# Autodesk Inventor assembly: Caster
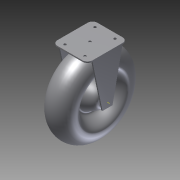
[picture p0: Inventor's stored thumbnail of the model, 180x180]
Saved by Autodesk Inventor 2012 (Build 160160000, 160)
## iProperties
Created: 2011-10-20
Part Number: Caster
Document SubType Name: Assembly
Designer: robotics
Author: robotics
## Documents named in this file (3)
- C:\Users\robotics\Dropbox\CAD Inventor\Preseason Projects\Cart Competition Cart\Team 2374\Caster.iam
- C:\Users\robotics\Dropbox\CAD Inventor\Preseason Projects\Cart Competition Cart\Team 2374\Caster2.ipt
- C:\Users\robotics\Dropbox\CAD Inventor\Preseason Projects\Cart Competition Cart\Team 2374\Wheel.ipt
## Components (2 placed, 2 different names)
1. Caster2:1 — Mate:1, Mate:2, Mate:3
2. Wheel:1 — Mate:1, Mate:2, Mate:3
## Relationships (3: Mate 3)
- Mate:1 (6.35 mm): Caster2:1 ↔ Wheel:1
- Mate:2 (107.95 mm): Caster2:1 ↔ Wheel:1
- Mate:3 (-50.8 mm): Caster2:1 ↔ Wheel:1
